# Autodesk Inventor assembly: Soquete para lâmpada E27 MT-2302 - DECORLUX
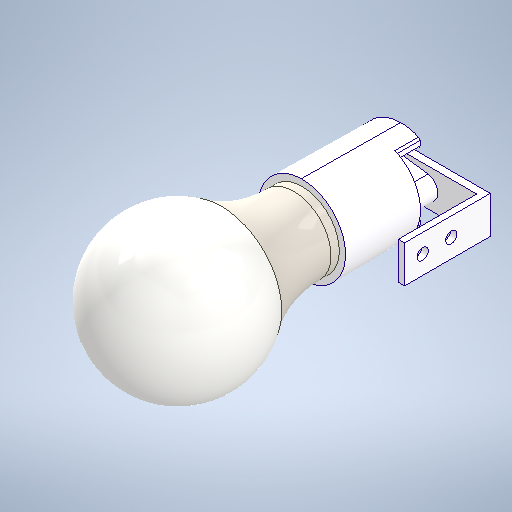
[picture p0: Inventor's stored thumbnail of the model, 512x512]
Saved by Autodesk Inventor 2025.1 (Build 291241000, 241)
## iProperties
Created: 2023-06-17
Part Number: Soquete para lâmpada E27 MT-2302 - DECORLUX
Description: STEP AP214
Document SubType Name: Assembly
Designer: pedro
Title: Soquete para lâmpada E27 MT-2302 - DECORLUX.STEP
Revision Number: ANY
Sending System: SolidWorks 2022
Preprocessor: SwSTEP 2.0
## Documents named in this file (5)
- C:\Users\pedro\Documents\1-CoisasSerias\UTFPR\2024-2\Oficina\Estrutura\Pecas Prontas\Let light\Soquete\Soquete para lâmpada E27 MT-2302 - DECORLUX\Soquete para lâmpada E27 MT-2302 - DECORLUX\Soquete para lâmpad.iam
- C:\Users\pedro\Documents\1-CoisasSerias\UTFPR\2024-2\Oficina\Estrutura\Pecas Prontas\Let light\Soquete\Soquete para lâmpada E27 MT-2302 - DECORLUX\Soquete para lâmpada E27 MT-2302 - DECORLUX\Cópia de copo porce.ipt
- C:\Users\pedro\Documents\1-CoisasSerias\UTFPR\2024-2\Oficina\Estrutura\Pecas Prontas\Let light\Soquete\Soquete para lâmpada E27 MT-2302 - DECORLUX\Soquete para lâmpada E27 MT-2302 - DECORLUX\Cópia de soquete E2.ipt
- C:\Users\pedro\Documents\1-CoisasSerias\UTFPR\2024-2\Oficina\Estrutura\Pecas Prontas\Let light\Soquete\Soquete para lâmpada E27 MT-2302 - DECORLUX\Soquete para lâmpada E27 MT-2302 - DECORLUX\Cópia de aba intern.ipt
- C:\Users\pedro\Documents\1-CoisasSerias\UTFPR\2024-2\Oficina\Estrutura\Pecas Prontas\Let light\LED Light Bulb\LED Light Bulb\LED Light Bulb.ipt
## Components (4 placed, 4 different names)
1. Cópia de copo porcelana^Soquete para lâmpada E27 MT-2302 - DECORLUX_Valor predeterminado<Como usinado>_1 — Coincidente:1, Coincidente:2
2. Cópia de soquete E27^Soquete para lâmpada E27 MT-2302 - DECORLUX_2
3. Cópia de aba interna E27^Soquete para lâmpada E27 MT-2302 - DECORLUX_Valor predeterminado<Como usinado>_3
4. LED Light Bulb:1 — Coincidente:1, Coincidente:2
## Relationships (2: Mate 2)
- Coincidente:1 [Mate]: Cópia de copo porcelana^Soquete para lâmpada E27 MT-2302 - DECORLUX_Valor predeterminado<Como usinado>_1 ↔ LED Light Bulb:1
- Coincidente:2 [Mate]: Cópia de copo porcelana^Soquete para lâmpada E27 MT-2302 - DECORLUX_Valor predeterminado<Como usinado>_1 ↔ LED Light Bulb:1
